# Autodesk Inventor assembly: ManganPitik
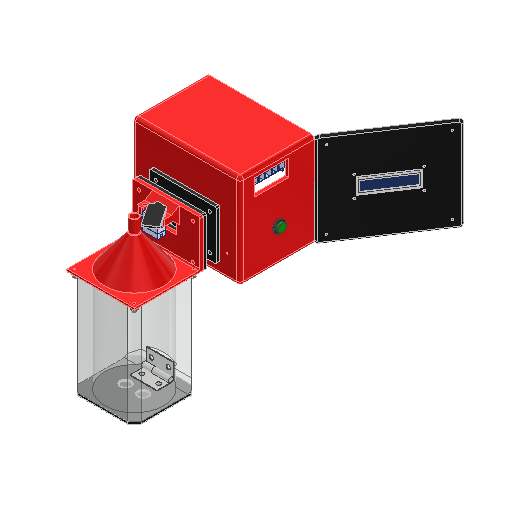
[picture p0: Inventor's stored thumbnail of the model, 512x512]
Saved by Autodesk Inventor 2026.2 (Build 302298010, 298A)
## iProperties
Created: 2026-05-22
Part Number: ManganPitik
Document SubType Name: Assembly
Designer: rizky
Author: rizky
## Documents named in this file (18)
- C:\SEMESTER 4\Mikrokontroller\PakanPitik\3D Design\ManganPitik.iam
- C:\SEMESTER 4\TEKNOFEST\Robolig\GripperGeser\servo-motor-sg90-mg90-1.snapshot.9\mg 90 micro servo\mg 90 micro servo\mg 90 micro servo.ipt
- C:\SEMESTER 4\Mikrokontroller\PakanPitik\3D Design\TutupTank.ipt
- C:\SEMESTER 4\Mikrokontroller\PakanPitik\3D Design\CorongBawah.ipt
- C:\SEMESTER 4\Mikrokontroller\PakanPitik\3D Design\Tank.ipt
- C:\SEMESTER 4\Mikrokontroller\PakanPitik\3D Design\TutupAtas.ipt
- C:\Bahan Commit\3D\hcsr-04-ultrasonic-sensor-1.snapshot.1\Ultrasonic HC-SR04\Ultrasonic HC-SR04\Ultrasonic HC-SR04.ipt
- C:\Bahan Commit\3D\hinges-1-1-2-inches-1.snapshot.4\Engsel 1 inch setengah\Engsel Female.ipt
- C:\Bahan Commit\3D\hinges-1-1-2-inches-1.snapshot.4\Engsel 1 inch setengah\Engsel Male.ipt
- C:\SEMESTER 4\Mikrokontroller\PakanPitik\3D Design\BracketPenghubung.ipt
- C:\Users\rizky\Downloads\.iam
- C:\Bahan Commit\3D\arduino-mega-2560-11.snapshot.1\Arduino Mega 2560 R3 v23\Arduino Mega 2560 R3 v23\Arduino Mega 2560 R3 v23.ipt
- C:\Users\rizky\Downloads\.ipt
- C:\Bahan Commit\3D\dc12v-5a-switching-power-supply-1.snapshot.1\12V-5A Model S\12V-5A Model S\12V-5A Model S.ipt
- C:\SEMESTER 4\Mikrokontroller\PakanPitik\3D Design\BoxIoT.ipt
- C:\SEMESTER 4\Mikrokontroller\PakanPitik\3D Design\TutupBox.ipt
- C:\Bahan Commit\3D\arduino-character-1602-16x2-lcd-display-module-i2c-3-3v-or-5v-1.snapshot.5\ERM1602-6\ERM1602-6\ERM1602-6.ipt
- C:\Bahan Commit\3D\panel-mount-push-button-switch-green-cap-1.snapshot.1\Push Button\STEP FILE\Push_Button\Push_Button\Push_Button.ipt
## Components (17 placed, 16 different names)
1. mg 90 micro servo:1 — Mate:5, Mate:6, Mate:7, Mate:8, Mate:9
2. CorongBawah:1 — Mate:5, Mate:8, Mate:9, Mate:10, Mate:11, Mate:12, Mate:47, Mate:48, Mate:49
3. TutupTank:1 — Mate:6, Mate:7
4. Tank:1 — Mate:10, Mate:11, Mate:12, Mate:41, Mate:42, Mate:43, Mate:76
5. TutupAtas:1 — Mate:31, Mate:34, Mate:38, Mate:44, Mate:45, Mate:46, Mate:76
6. Ultrasonic HC-SR04:1 — Mate:31, Mate:34, Mate:38
7. Engsel Female:1 — Mate:39, Mate:40, Mate:44, Mate:45, Mate:46
8. Engsel Male:1 — Mate:39, Mate:40, Mate:41, Mate:42, Mate:43
9. BracketPenghubung:1 — Mate:47, Mate:48, Mate:49, Mate:68, Mate:69, Mate:70
10. :1 [sub-assembly] — Mate:51, Mate:52, Mate:53
11. Arduino Mega 2560 R3 v23:1 — Mate:51, Mate:52, Mate:53, Mate:59, Mate:64
12. :2 — Mate:65, Mate:66, Mate:67
13. 12V-5A Model S:2 — Mate:61, Mate:62, Mate:63
14. BoxIoT:1 — Mate:59, Mate:61, Mate:62, Mate:63, Mate:64, Mate:65, Mate:66, Mate:67, Mate:68, Mate:69, Mate:70, Mate:77, Mate:78, Mate:79
15. TutupBox:1 — Mate:79, Mate:80, Mate:81, Mate:82
16. ERM1602-6:1 — Mate:80, Mate:81, Mate:82
17. Push_Button:1 — Mate:77, Mate:78
## Relationships (43: Mate 43)
- Mate:5: mg 90 micro servo:1 ↔ CorongBawah:1
- Mate:6: mg 90 micro servo:1 ↔ TutupTank:1
- Mate:7: mg 90 micro servo:1 ↔ TutupTank:1
- Mate:8: mg 90 micro servo:1 ↔ CorongBawah:1
- Mate:9: mg 90 micro servo:1 ↔ CorongBawah:1
- Mate:10: CorongBawah:1 ↔ Tank:1
- Mate:11: CorongBawah:1 ↔ Tank:1
- Mate:12: CorongBawah:1 ↔ Tank:1
- Mate:31: TutupAtas:1 ↔ Ultrasonic HC-SR04:1
- Mate:34: TutupAtas:1 ↔ Ultrasonic HC-SR04:1
- Mate:38: TutupAtas:1 ↔ Ultrasonic HC-SR04:1
- Mate:39: Engsel Female:1 ↔ Engsel Male:1
- Mate:40: Engsel Female:1 ↔ Engsel Male:1
- Mate:41: Tank:1 ↔ Engsel Male:1
- Mate:42: Tank:1 ↔ Engsel Male:1
- Mate:43: Tank:1 ↔ Engsel Male:1
- Mate:44: TutupAtas:1 ↔ Engsel Female:1
- Mate:45: TutupAtas:1 ↔ Engsel Female:1
- Mate:46: TutupAtas:1 ↔ Engsel Female:1
- Mate:47: CorongBawah:1 ↔ BracketPenghubung:1
- Mate:48: CorongBawah:1 ↔ BracketPenghubung:1
- Mate:49: CorongBawah:1 ↔ BracketPenghubung:1
- Mate:51: :1 ↔ Arduino Mega 2560 R3 v23:1
- Mate:52: :1 ↔ Arduino Mega 2560 R3 v23:1
- Mate:53: :1 ↔ Arduino Mega 2560 R3 v23:1
- Mate:59: Arduino Mega 2560 R3 v23:1 ↔ BoxIoT:1
- Mate:61: 12V-5A Model S:2 ↔ BoxIoT:1
- Mate:62: 12V-5A Model S:2 ↔ BoxIoT:1
- Mate:63: 12V-5A Model S:2 ↔ BoxIoT:1
- Mate:64: Arduino Mega 2560 R3 v23:1 ↔ BoxIoT:1
- Mate:65: :2 ↔ BoxIoT:1
- Mate:66: :2 ↔ BoxIoT:1
- Mate:67: :2 ↔ BoxIoT:1
- Mate:68: BracketPenghubung:1 ↔ BoxIoT:1
- Mate:69: BracketPenghubung:1 ↔ BoxIoT:1
- Mate:70: BracketPenghubung:1 ↔ BoxIoT:1
- Mate:76: Tank:1 ↔ TutupAtas:1
- Mate:77: BoxIoT:1 ↔ Push_Button:1
- Mate:78: BoxIoT:1 ↔ Push_Button:1
- Mate:79: BoxIoT:1 ↔ TutupBox:1
- Mate:80: TutupBox:1 ↔ ERM1602-6:1
- Mate:81: TutupBox:1 ↔ ERM1602-6:1
- Mate:82: TutupBox:1 ↔ ERM1602-6:1
